# Autodesk Inventor assembly: link9_SubAssembly.ipt
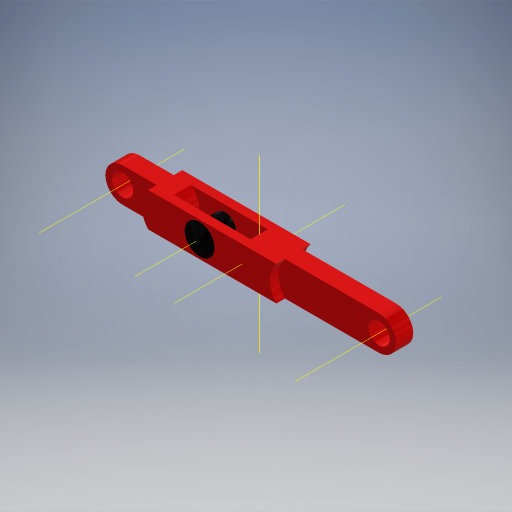
[picture p0: Inventor's stored thumbnail of the model, 512x512]
Saved by Autodesk Inventor 2024.2 (Build 282272000, 272)
## iProperties
Created: 2023-11-11
Part Number: link9_SubAssembly.ipt
Document SubType Name: Assembly
Designer: Camilo
Mass: 0.859144 g
Surface Area: 6.00448 cm^2
Volume: 0.318201 cm^3
Density: 2.7 g/cm^3
Author: Camilo
## Documents named in this file (3)
- D:\Documentos\MEGA\Universidad\2023-2\DinamicaComputacionalDeSistemasMulticuerpo\DinamicaComputacionalSistemasMulticuerpo\Proyecto\CAD\3D\link6_SubAssembly.iam
- D:\Documentos\MEGA\Universidad\2023-2\DinamicaComputacionalDeSistemasMulticuerpo\DinamicaComputacionalSistemasMulticuerpo\Proyecto\CAD\3D\link6.ipt
- D:\Documentos\MEGA\Universidad\2023-2\DinamicaComputacionalDeSistemasMulticuerpo\DinamicaComputacionalSistemasMulticuerpo\Proyecto\CAD\3D\bolt.ipt
## Components (2 placed, 2 different names)
1. link6:1 — Insert:1
2. bolt:1 — Insert:1
## Relationships (1: Insert 1)
- Insert:1: link6:1 ↔ bolt:1
